# Autodesk Inventor assembly: 21-30-101_ZI02 Grundgestell kpl-Novi PS-17-7-2025
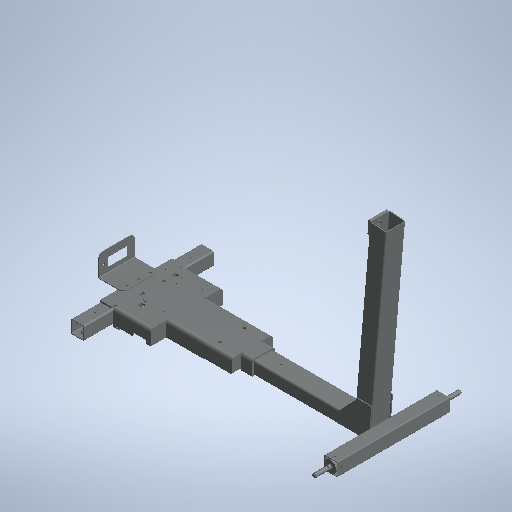
[picture p0: Inventor's stored thumbnail of the model, 512x512]
Saved by Autodesk Inventor 2025.2 (Build 292293000, 293)
## iProperties
Part Number: 21-30-101_ZI02 Grundgestell kpl-Novi PS-17-7-2025
Document SubType Name: Assembly
Designer: Zvonko.Gabric
Author: Zvonko.Gabric
## Documents named in this file (12)
- O:\Inventor SanaBike Series\SanaBike New PS\RACM\SB1000\Model\10-30-100 SanaBike 1000_RACM_550_PS_\10-30-100 SanaBike 1000_RACM_550_PS_\Sana bike 1000 ram sa novim PS (rupama,i prosirenjem)\21-30-101_ZI02 Grundgestell kpl-Novi PS-17-7-2025.iam
- O:\Inventor SanaBike Series\SanaBike New PS\RACM\SB1000\Model\10-30-100 SanaBike 1000_RACM_550_PS_\10-30-100 SanaBike 1000_RACM_550_PS_\Sana bike 1000 ram sa novim PS (rupama,i prosirenjem)\30-10-111_ZI03 Mittelrohr, Grundgestell.ipt
- O:\Inventor SanaBike Series\SanaBike New PS\RACM\SB1000\Model\10-30-100 SanaBike 1000_RACM_550_PS_\10-30-100 SanaBike 1000_RACM_550_PS_\21-30-102-A_ZI01 Querrohr vorne kpl, Grundgestell.iam
- O:\Inventor SanaBike Series\SanaBike New PS\RACM\SB1000\Model\10-30-100 SanaBike 1000_RACM_550_PS_\10-30-100 SanaBike 1000_RACM_550_PS_\Sana bike 1000 ram sa novim PS (rupama,i prosirenjem)\30-30-103_ZI01 Querrohr hinten, Grundgestell.ipt
- O:\Inventor SanaBike Series\SanaBike New PS\RACM\SB1000\Model\10-30-100 SanaBike 1000_RACM_550_PS_\10-30-100 SanaBike 1000_RACM_550_PS_\Sana bike 1000 ram sa novim PS (rupama,i prosirenjem)\28-30-100_ZI02 Winkelblech, Netzstecker.ipt
- O:\Inventor SanaBike Series\SanaBike New PS\RACM\SB1000\Model\10-30-100 SanaBike 1000_RACM_550_PS_\10-30-100 SanaBike 1000_RACM_550_PS_\31-10-114_ZI01 Versteifungsblech, Grundgestell.ipt
- O:\Inventor SanaBike Series\SanaBike New PS\RACM\SB1000\Model\10-30-100 SanaBike 1000_RACM_550_PS_\10-30-100 SanaBike 1000_RACM_550_PS_\31-10-112_ZI01 Versteifung, Mittelteilblech, Grundgestell.ipt
- O:\Inventor SanaBike Series\SanaBike New PS\RACM\SB1000\Model\10-30-100 SanaBike 1000_RACM_550_PS_\10-30-100 SanaBike 1000_RACM_550_PS_\Sana bike 1000 ram sa novim PS (rupama,i prosirenjem)\21-30-101-A_ZI04 Führungsrohr, Lenkerstange, kpl v3.iam
- O:\Inventor SanaBike Series\SanaBike New PS\RACM\SB1000\Model\10-30-100 SanaBike 1000_RACM_550_PS_\10-30-100 SanaBike 1000_RACM_550_PS_\Sana bike 1000 ram sa novim PS (rupama,i prosirenjem)\28-30-101-A1_ZI06 Mittelteilblech, Grundges.ipt
- O:\Inventor SanaBike Series\SanaBike New PS\RACM\SB1000\Model\10-30-100 SanaBike 1000_RACM_550_PS_\10-30-100 SanaBike 1000_RACM_550_PS_\Sana bike 1000 ram sa novim PS (rupama,i prosirenjem)\28-30-101-A2_ZI00 Blende1, Mittelteilblech, Grundgestell-.ipt
- O:\Inventor SanaBike Series\SanaBike New PS\RACM\SB1000\Model\10-30-100 SanaBike 1000_RACM_550_PS_\10-30-100 SanaBike 1000_RACM_550_PS_\Sana bike 1000 ram sa novim PS (rupama,i prosirenjem)\28-30-101-A3_ZI00 Blende2, Mittelteilblech, Grundgestell-.ipt
- C:\Users\Zvonko.Gabric.GANSHORN\Desktop\SanaBike\SanaBike 1000\10-30-100 SanaBike 1000_\10-30-100 SanaBike 1000_\28-30-101-A6_ZI00 Gewindebolzen, Netzteilplatine, Grundgestell-.ipt
## Components (17 placed, 11 different names)
1. 30-10-111_ZI03 Mittelrohr, Grundgestell:1 — Mate:1, Mate:4, Mate:5
2. 28-30-101-A1_ZI06 Mittelteilblech, Grundges:1 — Mate:4, Flush:1, Mate:5, Mate:12, Tangent:1
3. 21-30-102-A_ZI01 Querrohr vorne kpl, Grundgestell:1 [sub-assembly]
4. 30-30-103_ZI01 Querrohr hinten, Grundgestell:1 — Flush:1
5. 28-30-100_ZI02 Winkelblech, Netzstecker:1
6. 31-10-114_ZI01 Versteifungsblech, Grundgestell:1 — Mate:2
7. 31-10-114_ZI01 Versteifungsblech, Grundgestell:2 — Mate:3
8. 31-10-112_ZI01 Versteifung, Mittelteilblech, Grundgestell:1
9. 21-30-101-A_ZI04 Führungsrohr, Lenkerstange, kpl v3:1 [sub-assembly] — Mate:1, Mate:2, Mate:3
10. 28-30-101-A2_ZI00 Blende1, Mittelteilblech, Grundgestell-:1
11. 28-30-101-A2_ZI00 Blende1, Mittelteilblech, Grundgestell-:2 — Tangent:2
12. 28-30-101-A3_ZI00 Blende2, Mittelteilblech, Grundgestell-:1
13. 28-30-101-A3_ZI00 Blende2, Mittelteilblech, Grundgestell-:2
14. 28-30-101-A6_ZI00 Gewindebolzen, Netzteilplatine, Grundgestell-:1 — Mate:12, Tangent:1, Tangent:2
15. 28-30-101-A6_ZI00 Gewindebolzen, Netzteilplatine, Grundgestell-:2
16. 28-30-101-A6_ZI00 Gewindebolzen, Netzteilplatine, Grundgestell-:3
17. 28-30-101-A6_ZI00 Gewindebolzen, Netzteilplatine, Grundgestell-:4
## Component patterns: (4 elements, first: 28-30-101-A6_ZI00 Gewindebolzen, Netzteilplatine, Grundgestell-:1)
## Relationships (17: Mate 12, Flush 3, Tangent 2)
- Mate:1: 30-10-111_ZI03 Mittelrohr, Grundgestell:1 ↔ 21-30-101-A_ZI04 Führungsrohr, Lenkerstange, kpl v3:1
- Mate:2: 31-10-114_ZI01 Versteifungsblech, Grundgestell:1 ↔ 21-30-101-A_ZI04 Führungsrohr, Lenkerstange, kpl v3:1
- Mate:3: 31-10-114_ZI01 Versteifungsblech, Grundgestell:2 ↔ 21-30-101-A_ZI04 Führungsrohr, Lenkerstange, kpl v3:1
- Mate:4: 30-10-111_ZI03 Mittelrohr, Grundgestell:1 ↔ 28-30-101-A1_ZI06 Mittelteilblech, Grundges:1
- Flush:1: 28-30-101-A1_ZI06 Mittelteilblech, Grundges:1 ↔ 30-30-103_ZI01 Querrohr hinten, Grundgestell:1
- Mate:5: 30-10-111_ZI03 Mittelrohr, Grundgestell:1 ↔ 28-30-101-A1_ZI06 Mittelteilblech, Grundges:1
- [Mate]: 28-30-101-A1_ZI06 Mittelteilblech, Grundges:1 ↔ 28-30-101-A2_ZI00 Blende1, Mittelteilblech, Grundgestell-:1
- [Flush]: 28-30-101-A1_ZI06 Mittelteilblech, Grundges:1 ↔ 28-30-101-A2_ZI00 Blende1, Mittelteilblech, Grundgestell-:1
- [Mate]: 28-30-101-A1_ZI06 Mittelteilblech, Grundges:1 ↔ 28-30-101-A2_ZI00 Blende1, Mittelteilblech, Grundgestell-:1
- [Mate]: 28-30-101-A1_ZI06 Mittelteilblech, Grundges:1 ↔ 28-30-101-A2_ZI00 Blende1, Mittelteilblech, Grundgestell-:2
- [Flush]: 28-30-101-A1_ZI06 Mittelteilblech, Grundges:1 ↔ 28-30-101-A2_ZI00 Blende1, Mittelteilblech, Grundgestell-:2
- [Mate]: 28-30-101-A1_ZI06 Mittelteilblech, Grundges:1 ↔ 28-30-101-A2_ZI00 Blende1, Mittelteilblech, Grundgestell-:2
- [Mate]: 28-30-101-A1_ZI06 Mittelteilblech, Grundges:1 ↔ 28-30-101-A3_ZI00 Blende2, Mittelteilblech, Grundgestell-:1
- [Mate]: 28-30-101-A1_ZI06 Mittelteilblech, Grundges:1 ↔ 28-30-101-A3_ZI00 Blende2, Mittelteilblech, Grundgestell-:2
- Mate:12: 28-30-101-A1_ZI06 Mittelteilblech, Grundges:1 ↔ 28-30-101-A6_ZI00 Gewindebolzen, Netzteilplatine, Grundgestell-:1
- Tangent:1 (8.5 mm): 28-30-101-A1_ZI06 Mittelteilblech, Grundges:1 ↔ 28-30-101-A6_ZI00 Gewindebolzen, Netzteilplatine, Grundgestell-:1
- Tangent:2 (-11.5 mm): 28-30-101-A2_ZI00 Blende1, Mittelteilblech, Grundgestell-:2 ↔ 28-30-101-A6_ZI00 Gewindebolzen, Netzteilplatine, Grundgestell-:1
